# Autodesk Inventor assembly: ViseBAssembly
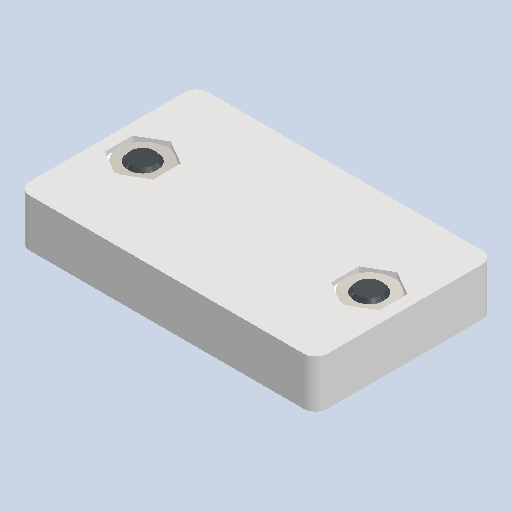
[picture p0: Inventor's stored thumbnail of the model, 512x512]
Saved by Autodesk Inventor 2022 (Build 260153000, 153)
## iProperties
Created: 2021-11-10
Part Number: ViseBAssembly
Document SubType Name: Assembly
Designer: JK
Author: JK
## Documents named in this file (4)
- C:\Users\JK\Documents\Inventor\UTM\ViseBAssembly.iam
- C:\Users\JK\Documents\Inventor\UTM\ViseB.ipt
- C:\Users\JK\Documents\Inventor\UTM\M5Nut.ipt
- C:\Users\JK\Documents\Inventor\UTM\PernoM5x8Plano.ipt
## Components (5 placed, 3 different names)
1. ViseB:1
2. M5Nut:1
3. M5Nut:2
4. PernoM5x8Plano:1
5. PernoM5x8Plano:2
## Relationships (10: Mate 7, Angle 2, Flush 1)
- [Mate]: ViseB:1 ↔ M5Nut:1
- [Angle] (0 deg): ViseB:1 ↔ M5Nut:1
- [Mate]: ViseB:1 ↔ M5Nut:1
- [Mate]: ViseB:1 ↔ M5Nut:2
- [Angle] (0 deg): ViseB:1 ↔ M5Nut:2
- [Mate]: ViseB:1 ↔ M5Nut:2
- [Mate]: ViseB:1 ↔ PernoM5x8Plano:2
- [Mate]: ViseB:1 ↔ PernoM5x8Plano:1
- [Mate]: ViseB:1 ↔ PernoM5x8Plano:2
- [Flush]: PernoM5x8Plano:1 ↔ PernoM5x8Plano:2
